# Autodesk Inventor assembly: rev2 base
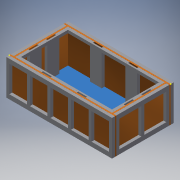
[picture p0: Inventor's stored thumbnail of the model, 180x180]
Saved by Autodesk Inventor 2017 (Build 210142000, 142)
## iProperties
Created: 2019-05-04
Part Number: rev2 base
Document SubType Name: Assembly
Designer: Roman
Author: Roman
## Documents named in this file (4)
- C:\Users\Roman\Documents\CAD\enclosure rev1\rev2 base\rev2 base.iam
- C:\Users\Roman\Documents\CAD\enclosure rev1\rev2 base\rev1 large wall\rev1 base large wall.iam
- C:\Users\Roman\Documents\CAD\enclosure rev1\rev2 base\rev1 small wall\rev1 base short wall.iam
- C:\Users\Roman\Documents\CAD\enclosure rev1\rev2 base\rev1 base floor.ipt
## Components (5 placed, 3 different names)
1. rev1 base large wall:1 [sub-assembly] — Mate:1, Flush:1, Flush:2, Flush:5, Mate:3, Flush:10
2. rev1 base short wall:1 [sub-assembly] — Mate:1, Flush:1, Flush:2
3. rev1 base short wall:2 [sub-assembly] — Flush:5, Mate:3, Flush:8, Mate:5, Flush:9, Flush:10, Mate:6, Flush:11
4. rev1 base large wall:2 [sub-assembly] — Flush:8, Mate:5, Flush:9, Mate:7
5. rev1 base floor:1 — Mate:6, Flush:11, Mate:7
## Relationships (12: Flush 7, Mate 5)
- Mate:1: rev1 base large wall:1 ↔ rev1 base short wall:1
- Flush:1: rev1 base large wall:1 ↔ rev1 base short wall:1
- Flush:2: rev1 base large wall:1 ↔ rev1 base short wall:1
- Flush:5: rev1 base large wall:1 ↔ rev1 base short wall:2
- Mate:3: rev1 base large wall:1 ↔ rev1 base short wall:2
- Flush:8: rev1 base short wall:2 ↔ rev1 base large wall:2
- Mate:5: rev1 base short wall:2 ↔ rev1 base large wall:2
- Flush:9: rev1 base short wall:2 ↔ rev1 base large wall:2
- Flush:10: rev1 base large wall:1 ↔ rev1 base short wall:2
- Mate:6: rev1 base short wall:2 ↔ rev1 base floor:1
- Flush:11: rev1 base short wall:2 ↔ rev1 base floor:1
- Mate:7: rev1 base large wall:2 ↔ rev1 base floor:1
